# Autodesk Inventor assembly: Assembly_miniSPIM_v0
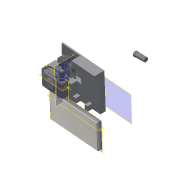
[picture p0: Inventor's stored thumbnail of the model, 180x180]
Saved by Autodesk Inventor 2019 (Build 230136000, 136)
## iProperties
Created: 2019-07-21
Part Number: Assembly_miniSPIM_v0
Document SubType Name: Assembly
Designer: diederichbenedict
Author: diederichbenedict
## Documents named in this file (11)
- C:\Users\diederichbenedict\Dropbox\Dokumente\Promotion\PROJECTS\miniSPIM\INVENTOR\Assembly_miniSPIM_v0.iam
- C:\Users\diederichbenedict\Dropbox\Dokumente\Promotion\PROJECTS\miniSPIM\INVENTOR\100_DXO_Camera v2.ipt
- C:\Users\diederichbenedict\Dropbox\Dokumente\Promotion\PROJECTS\miniSPIM\INVENTOR\101_CCTV_Lens_Thread.ipt
- C:\Users\diederichbenedict\Dropbox\Dokumente\Promotion\PROJECTS\miniSPIM\INVENTOR\103_CCTV_Lens_f2.8_f#1.ipt
- C:\Users\diederichbenedict\Dropbox\Dokumente\Promotion\PROJECTS\miniSPIM\INVENTOR\104_CCTV_Lens_f2.8_#1.ipt
- C:\Users\diederichbenedict\Dropbox\Dokumente\Promotion\PROJECTS\miniSPIM\INVENTOR\109_Chinese_XY_stage.ipt
- C:\Users\diederichbenedict\Dropbox\Dokumente\Promotion\PROJECTS\miniSPIM\INVENTOR\00_Sony_MDL_Projector.ipt
- C:\Users\diederichbenedict\Dropbox\Dokumente\Promotion\PROJECTS\miniSPIM\INVENTOR\10_Baseplate_Minispim.ipt
- C:\Users\diederichbenedict\Dropbox\Dokumente\Promotion\PROJECTS\miniSPIM\INVENTOR\10_Lidplate_Minispim.ipt
- C:\Users\diederichbenedict\Dropbox\Dokumente\Promotion\PROJECTS\miniSPIM\INVENTOR\00_Lens_f_25mm.ipt
- C:\Users\diederichbenedict\Dropbox\Dokumente\Promotion\PROJECTS\miniSPIM\INVENTOR\10_Lid_Minispim.ipt
## Components (10 placed, 10 different names)
1. 100_DXO_Camera v2:1 — Insert:2, Mate:6, Mate:14, Flush:9
2. 103_CCTV_Lens_f2.8_f#1:1 — Insert:2, Insert:4, Mate:9, Mate:10
3. 104_CCTV_Lens_f2.8_#1:1
4. 101_CCTV_Lens_Thread:2 — Insert:4
5. 10_Baseplate_Minispim:1 — Flush:6, Flush:7, Mate:14, Flush:8
6. 109_Chinese_XY_stage:1 — Mate:6
7. 10_Lidplate_Minispim:1 — Flush:6, Flush:7
8. 00_Lens_f_25mm:1
9. 10_Lid_Minispim:1 — Flush:8
10. 00_Sony_MDL_Projector:1 — Flush:9
## Relationships (11: Mate 5, Flush 4, Insert 2)
- Insert:2 (-2 mm): 100_DXO_Camera v2:1 ↔ 103_CCTV_Lens_f2.8_f#1:1
- Insert:4 (5 mm): 103_CCTV_Lens_f2.8_f#1:1 ↔ 101_CCTV_Lens_Thread:2
- Mate:6 (8 mm): 100_DXO_Camera v2:1 ↔ 109_Chinese_XY_stage:1
- Flush:6: 10_Baseplate_Minispim:1 ↔ 10_Lidplate_Minispim:1
- Flush:7: 10_Baseplate_Minispim:1 ↔ 10_Lidplate_Minispim:1
- Mate:9: 103_CCTV_Lens_f2.8_f#1:1
- Mate:10: 103_CCTV_Lens_f2.8_f#1:1
- Mate:11
- Mate:14: 100_DXO_Camera v2:1 ↔ 10_Baseplate_Minispim:1
- Flush:8: 10_Baseplate_Minispim:1 ↔ 10_Lid_Minispim:1
- Flush:9: 100_DXO_Camera v2:1 ↔ 00_Sony_MDL_Projector:1
